# Autodesk Inventor assembly: finales Ruder mit plattform
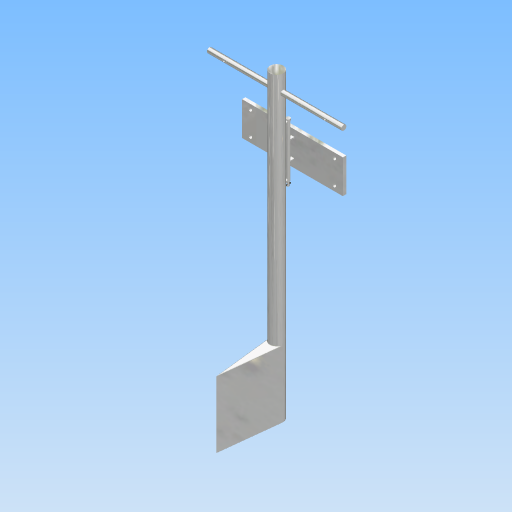
[picture p0: Inventor's stored thumbnail of the model, 512x512]
Saved by Autodesk Inventor 2024.4 (Build 284460000, 460)
## iProperties
Created: 2026-01-22
Part Number: finales Ruder mit plattform
Document SubType Name: Assembly
Designer: lucas
Mass: 2105.37 g
Surface Area: 2859.22 cm^2
Volume: 2104.76 cm^3
Density: 1.00029 g/cm^3
## Documents named in this file (5)
- C:\Users\windows-desktop\Desktop\Studium\Konstruktion\VaultWorkspace\Daten\I60-Konstruktion\I60-Gruppe-4\Bluhm\Daten\I60-Konstruktion\I60-Gruppe-4\Bluhm\Ruder\finales_Ruder_mit_Plattform.iam
- C:\Users\windows-desktop\Desktop\Studium\Konstruktion\VaultWorkspace\Daten\I60-Konstruktion\I60-Gruppe-4\Bluhm\Daten\I60-Konstruktion\I60-Gruppe-4\David\Ruder bündig.iam
- C:\Users\windows-desktop\Desktop\Studium\Konstruktion\VaultWorkspace\Daten\I60-Konstruktion\I60-Gruppe-4\Bluhm\Daten\I60-Konstruktion\I60-Gruppe-4\David\Plattform mit Rohr für Montierung.ipt
- C:\Users\windows-desktop\Desktop\Studium\Konstruktion\VaultWorkspace\Daten\I60-Konstruktion\I60-Gruppe-4\Bluhm\Daten\I60-Konstruktion\I60-Gruppe-4\David\Bolzen fuer Ruder.ipt
- C:\Users\windows-desktop\Desktop\Studium\Konstruktion\VaultWorkspace\Daten\I60-Konstruktion\I60-Gruppe-4\Bluhm\Normteile\de-DE\ISO 1234(1)\ISO 1234 - 2,5 x 12DIN EN.ipt
## Components (4 placed, 4 different names)
1. Ruder bündig:1 [sub-assembly] — Einfügen:1, Einfügen:2
2. Plattform mit Rohr für Montierung:1 — Einfügen:1
3. Bolzen fuer Ruder:1 — Einfügen:2, Passend:1
4. DIN EN ISO 1234 2,5 x 12:1 — Passend:1
## Relationships (3: Insert 2, Mate 1)
- Einfügen:1 [Insert]: Ruder bündig:1 ↔ Plattform mit Rohr für Montierung:1
- Einfügen:2 [Insert]: Ruder bündig:1 ↔ Bolzen fuer Ruder:1
- Passend:1 [Mate]: Bolzen fuer Ruder:1 ↔ DIN EN ISO 1234 2,5 x 12:1
